# Autodesk Inventor assembly: Klapp-Baugruppe_für_Antrieb
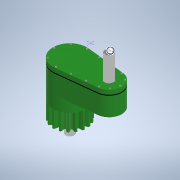
[picture p0: Inventor's stored thumbnail of the model, 180x180]
Saved by Autodesk Inventor 2021 (Build 250183000, 183)
## iProperties
Created: 2021-01-12
Part Number: Klapp-Baugruppe_für_Antrieb
Document SubType Name: Assembly
Designer: Jaro Machnow
Author: Jaro Machnow
## Documents named in this file (11)
- C:\Users\Jaro Machnow\Documents\Vault\Gruppen\Gruppe 2\Entwurf\Amphibienfahrzeug\Wechsel zwischen Land und Wasser\Wechselmechanik\Klappmechanismus\Klapp-Baugruppe_für_Antrieb.iam
- C:\Users\Jaro Machnow\Documents\Vault\Gruppen\Gruppe 2\Entwurf\Amphibienfahrzeug\Wechsel zwischen Land und Wasser\Wechselmechanik\Klappmechanismus\Klapp_Welle_zur_Karosserie.ipt
- C:\Users\Jaro Machnow\Documents\Vault\Gruppen\Gruppe 2\Entwurf\Amphibienfahrzeug\Wechsel zwischen Land und Wasser\Wechselmechanik\Klappmechanismus\Klapp_ Kraftübertragung mit Keilriemen.iam
- C:\Users\Jaro Machnow\Documents\Vault\Gruppen\Gruppe 2\Entwurf\Amphibienfahrzeug\Wechsel zwischen Land und Wasser\Wechselmechanik\Klappmechanismus\Klapp_Hinten_Welle_zum_Rad.ipt
- C:\Users\Jaro Machnow\Documents\Vault\Gruppen\Gruppe 2\Entwurf\Amphibienfahrzeug\Wechsel zwischen Land und Wasser\Wechselmechanik\Klappmechanismus\Klapp_Lager.iam
- C:\Users\Jaro Machnow\Documents\Vault\Gruppen\Gruppe 2\Entwurf\Amphibienfahrzeug\Wechsel zwischen Land und Wasser\Wechselmechanik\Klappmechanismus\Keilverbindung1.iam
- C:\Users\Jaro Machnow\Documents\Vault\Gruppen\Gruppe 2\Entwurf\Amphibienfahrzeug\Wechsel zwischen Land und Wasser\Wechselmechanik\Klappmechanismus\Keilverbindung2.iam
- C:\Users\Jaro Machnow\Documents\Vault\Gruppen\Gruppe 2\Entwurf\Amphibienfahrzeug\Wechsel zwischen Land und Wasser\Wechselmechanik\Klappmechanismus\Klapp_Dichtungsgummi.ipt
- C:\Users\Jaro Machnow\Documents\Vault\Gruppen\Gruppe 2\Entwurf\Amphibienfahrzeug\Wechsel zwischen Land und Wasser\Wechselmechanik\Klappmechanismus\Klapp_Hinten_Abdeckung.ipt
- C:\Users\Jaro Machnow\Documents\Vault\Gruppen\Gruppe 2\Entwurf\Amphibienfahrzeug\Wechsel zwischen Land und Wasser\Wechselmechanik\Klappmechanismus\Klapphülle_neu.ipt
- C:\Users\Jaro Machnow\Documents\Inventor\Content Center Files\R2021\de-DE\DIN 84\DIN 84 - M1 x 10.ipt
## Components (26 placed, 8 different names)
1. Welle:1 — Fluchtend:2, Passend:5, Fluchtend:6, Passend:10, Passend:11, Passend:12, Winkel:2, Passend:31, Passend:32, Passend:33, Fluchtend:7, Winkel:5, Passend:69
2. Kraftübertragung mit Keilriemen:1 [sub-assembly] — Passend:3, Passend:10, Winkel:2, Winkel:4, Passend:32
3. Welle:2 — Passend:3, Fluchtend:2, Passend:8, Passend:9, Winkel:4, Passend:18, Passend:19, Passend:40, Passend:70, Winkel:6, Passend:71
4. Lager:1 [sub-assembly] — Passend:5, Fluchtend:6, Passend:34
5. Lager:2 [sub-assembly] — Passend:8, Passend:9
6. Lager:3 [sub-assembly] — Passend:11, Passend:12
7. Keilverbindung:1 [sub-assembly] — Fluchtend:7, Winkel:5, Passend:69
8. Keilverbindung:2 [sub-assembly] — Passend:70, Winkel:6, Passend:71
9. Lager:4 [sub-assembly] — Passend:18, Passend:19
10. Klapp_Dichtungsgummi:1 — Passend:25, Passend:26, Passend:35, Passend:36, Passend:38
11. Klapp_Hinten_Abdeckung:1 — Passend:25, Passend:26, Passend:31, Passend:37, Passend:39, Passend:41, Passend:42, Passend:43, Passend:44, Passend:45, Passend:46, Passend:47, Passend:48, Passend:49, Passend:50, Passend:51, Passend:52, Passend:53, Passend:54, Passend:55, Passend:56, Passend:57, Passend:58, Passend:59, Passend:60, Passend:61, Passend:62, Passend:63, Passend:64, Passend:65, Passend:66, Passend:67, Passend:68
12. Klapphülle_neu:1 — Passend:33, Passend:34, Passend:35, Passend:36, Passend:37, Passend:38, Passend:39, Passend:40
13. DIN 84 - ersetzt durch DIN EN ISO 1207 M1 x 10:1 — Passend:41, Passend:42
14. DIN 84 - ersetzt durch DIN EN ISO 1207 M1 x 10:2 — Passend:43, Passend:44
15. DIN 84 - ersetzt durch DIN EN ISO 1207 M1 x 10:3 — Passend:45, Passend:46
16. DIN 84 - ersetzt durch DIN EN ISO 1207 M1 x 10:4 — Passend:47, Passend:48
17. DIN 84 - ersetzt durch DIN EN ISO 1207 M1 x 10:5 — Passend:49, Passend:50
18. DIN 84 - ersetzt durch DIN EN ISO 1207 M1 x 10:6 — Passend:51, Passend:52
19. DIN 84 - ersetzt durch DIN EN ISO 1207 M1 x 10:7 — Passend:53, Passend:54
20. DIN 84 - ersetzt durch DIN EN ISO 1207 M1 x 10:8 — Passend:55, Passend:56
21. DIN 84 - ersetzt durch DIN EN ISO 1207 M1 x 10:9 — Passend:57, Passend:58
22. DIN 84 - ersetzt durch DIN EN ISO 1207 M1 x 10:10 — Passend:59, Passend:60
23. DIN 84 - ersetzt durch DIN EN ISO 1207 M1 x 10:11 — Passend:61, Passend:62
24. DIN 84 - ersetzt durch DIN EN ISO 1207 M1 x 10:12 — Passend:63, Passend:64
25. DIN 84 - ersetzt durch DIN EN ISO 1207 M1 x 10:13 — Passend:65, Passend:66
26. DIN 84 - ersetzt durch DIN EN ISO 1207 M1 x 10:14 — Passend:67, Passend:68
## Relationships (59: Mate 52, Angle 4, Flush 3)
- Passend:3 [Mate]: Kraftübertragung mit Keilriemen:1 ↔ Welle:2
- Fluchtend:2 [Flush]: Welle:1 ↔ Welle:2
- Passend:5 [Mate]: Welle:1 ↔ Lager:1
- Fluchtend:6 [Flush]: Welle:1 ↔ Lager:1
- Passend:8 [Mate]: Welle:2 ↔ Lager:2
- Passend:9 [Mate]: Welle:2 ↔ Lager:2
- Passend:10 [Mate]: Welle:1 ↔ Kraftübertragung mit Keilriemen:1
- Passend:11 [Mate]: Welle:1 ↔ Lager:3
- Passend:12 [Mate]: Welle:1 ↔ Lager:3
- Winkel:2 [Angle] (174.2383 deg): Welle:1 ↔ Kraftübertragung mit Keilriemen:1
- Winkel:4 [Angle] (146.2544 deg): Kraftübertragung mit Keilriemen:1 ↔ Welle:2
- Passend:18 [Mate]: Welle:2 ↔ Lager:4
- Passend:19 [Mate]: Welle:2 ↔ Lager:4
- Passend:25 [Mate]: Klapp_Dichtungsgummi:1 ↔ Klapp_Hinten_Abdeckung:1
- Passend:26 [Mate]: Klapp_Dichtungsgummi:1 ↔ Klapp_Hinten_Abdeckung:1
- Passend:31 [Mate]: Welle:1 ↔ Klapp_Hinten_Abdeckung:1
- Passend:32 [Mate]: Welle:1 ↔ Kraftübertragung mit Keilriemen:1
- Passend:33 [Mate]: Welle:1 ↔ Klapphülle_neu:1
- Passend:34 [Mate]: Lager:1 ↔ Klapphülle_neu:1
- Passend:35 [Mate]: Klapp_Dichtungsgummi:1 ↔ Klapphülle_neu:1
- Passend:36 [Mate]: Klapp_Dichtungsgummi:1 ↔ Klapphülle_neu:1
- Passend:37 [Mate]: Klapp_Hinten_Abdeckung:1 ↔ Klapphülle_neu:1
- Passend:38 [Mate]: Klapp_Dichtungsgummi:1 ↔ Klapphülle_neu:1
- Passend:39 [Mate]: Klapp_Hinten_Abdeckung:1 ↔ Klapphülle_neu:1
- Passend:40 [Mate] (0.166 mm): Welle:2 ↔ Klapphülle_neu:1
- Passend:41 [Mate]: Klapp_Hinten_Abdeckung:1 ↔ DIN 84 - ersetzt durch DIN EN ISO 1207 M1 x 10:1
- Passend:42 [Mate]: Klapp_Hinten_Abdeckung:1 ↔ DIN 84 - ersetzt durch DIN EN ISO 1207 M1 x 10:1
- Passend:43 [Mate]: Klapp_Hinten_Abdeckung:1 ↔ DIN 84 - ersetzt durch DIN EN ISO 1207 M1 x 10:2
- Passend:44 [Mate]: Klapp_Hinten_Abdeckung:1 ↔ DIN 84 - ersetzt durch DIN EN ISO 1207 M1 x 10:2
- Passend:45 [Mate]: Klapp_Hinten_Abdeckung:1 ↔ DIN 84 - ersetzt durch DIN EN ISO 1207 M1 x 10:3
- Passend:46 [Mate]: Klapp_Hinten_Abdeckung:1 ↔ DIN 84 - ersetzt durch DIN EN ISO 1207 M1 x 10:3
- Passend:47 [Mate]: Klapp_Hinten_Abdeckung:1 ↔ DIN 84 - ersetzt durch DIN EN ISO 1207 M1 x 10:4
- Passend:48 [Mate]: Klapp_Hinten_Abdeckung:1 ↔ DIN 84 - ersetzt durch DIN EN ISO 1207 M1 x 10:4
- Passend:49 [Mate]: Klapp_Hinten_Abdeckung:1 ↔ DIN 84 - ersetzt durch DIN EN ISO 1207 M1 x 10:5
- Passend:50 [Mate]: Klapp_Hinten_Abdeckung:1 ↔ DIN 84 - ersetzt durch DIN EN ISO 1207 M1 x 10:5
- Passend:51 [Mate]: Klapp_Hinten_Abdeckung:1 ↔ DIN 84 - ersetzt durch DIN EN ISO 1207 M1 x 10:6
- Passend:52 [Mate]: Klapp_Hinten_Abdeckung:1 ↔ DIN 84 - ersetzt durch DIN EN ISO 1207 M1 x 10:6
- Passend:53 [Mate]: Klapp_Hinten_Abdeckung:1 ↔ DIN 84 - ersetzt durch DIN EN ISO 1207 M1 x 10:7
- Passend:54 [Mate]: Klapp_Hinten_Abdeckung:1 ↔ DIN 84 - ersetzt durch DIN EN ISO 1207 M1 x 10:7
- Passend:55 [Mate]: Klapp_Hinten_Abdeckung:1 ↔ DIN 84 - ersetzt durch DIN EN ISO 1207 M1 x 10:8
- Passend:56 [Mate]: Klapp_Hinten_Abdeckung:1 ↔ DIN 84 - ersetzt durch DIN EN ISO 1207 M1 x 10:8
- Passend:57 [Mate]: Klapp_Hinten_Abdeckung:1 ↔ DIN 84 - ersetzt durch DIN EN ISO 1207 M1 x 10:9
- Passend:58 [Mate]: Klapp_Hinten_Abdeckung:1 ↔ DIN 84 - ersetzt durch DIN EN ISO 1207 M1 x 10:9
- Passend:59 [Mate]: Klapp_Hinten_Abdeckung:1 ↔ DIN 84 - ersetzt durch DIN EN ISO 1207 M1 x 10:10
- Passend:60 [Mate]: Klapp_Hinten_Abdeckung:1 ↔ DIN 84 - ersetzt durch DIN EN ISO 1207 M1 x 10:10
- Passend:61 [Mate]: Klapp_Hinten_Abdeckung:1 ↔ DIN 84 - ersetzt durch DIN EN ISO 1207 M1 x 10:11
- Passend:62 [Mate]: Klapp_Hinten_Abdeckung:1 ↔ DIN 84 - ersetzt durch DIN EN ISO 1207 M1 x 10:11
- Passend:63 [Mate]: Klapp_Hinten_Abdeckung:1 ↔ DIN 84 - ersetzt durch DIN EN ISO 1207 M1 x 10:12
- Passend:64 [Mate]: Klapp_Hinten_Abdeckung:1 ↔ DIN 84 - ersetzt durch DIN EN ISO 1207 M1 x 10:12
- Passend:65 [Mate]: Klapp_Hinten_Abdeckung:1 ↔ DIN 84 - ersetzt durch DIN EN ISO 1207 M1 x 10:13
- Passend:66 [Mate]: Klapp_Hinten_Abdeckung:1 ↔ DIN 84 - ersetzt durch DIN EN ISO 1207 M1 x 10:13
- Passend:67 [Mate]: Klapp_Hinten_Abdeckung:1 ↔ DIN 84 - ersetzt durch DIN EN ISO 1207 M1 x 10:14
- Passend:68 [Mate]: Klapp_Hinten_Abdeckung:1 ↔ DIN 84 - ersetzt durch DIN EN ISO 1207 M1 x 10:14
- Fluchtend:7 [Flush] (1.0188 mm): Welle:1 ↔ Keilverbindung:1
- Winkel:5 [Angle] (0 deg): Welle:1 ↔ Keilverbindung:1
- Passend:69 [Mate]: Welle:1 ↔ Keilverbindung:1
- Passend:70 [Mate] (0.9486 mm): Welle:2 ↔ Keilverbindung:2
- Winkel:6 [Angle] (40 deg): Welle:2 ↔ Keilverbindung:2
- Passend:71 [Mate]: Welle:2 ↔ Keilverbindung:2
